# Autodesk Inventor assembly: Assembly6
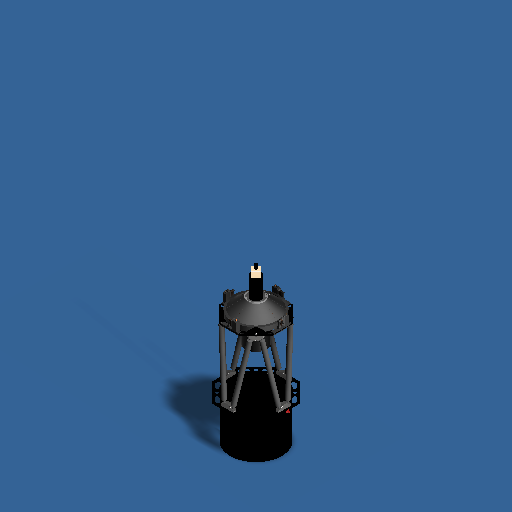
[picture p0: Inventor's stored thumbnail of the model, 512x512]
Saved by Autodesk Inventor 2026.2 (Build 302298000, 298)
## iProperties
Created: 2025-12-09
Part Number: Assembly6
Document SubType Name: Assembly
Designer: Thoma
Mass: 27295.5 g
Surface Area: 25498 cm^2
Volume: 10830.6 cm^3
Density: 2.52023 g/cm^3
Author: Thoma
## Documents named in this file (26)
- C:\Users\Thoma\OneDrive\Desktop\dir\telescope_cover\main\version_2\Main_v4.iam
- C:\Users\Thoma\OneDrive\Desktop\dir\telescope_cover\telescope\version_3\Telescope_End.ipt
- C:\Users\Thoma\OneDrive\Desktop\dir\telescope_cover\telescope\version_3\Triangle.ipt
- C:\Users\Thoma\OneDrive\Desktop\dir\telescope_cover\telescope\version_3\Triangle_Bracket_Top.ipt
- C:\Users\Thoma\OneDrive\Desktop\dir\telescope_cover\telescope\version_3\Carbon_Fibre.ipt
- C:\Users\Thoma\OneDrive\Desktop\dir\telescope_cover\telescope\version_3\5mm Screw.ipt
- C:\Users\Thoma\OneDrive\Desktop\dir\telescope_cover\telescope\version_3\35mm_bolt.ipt
- C:\Users\Thoma\OneDrive\Desktop\dir\telescope_cover\telescope\version_3\Triangle_Bracket_Bottom_MIR.ipt
- C:\Users\Thoma\OneDrive\Desktop\dir\telescope_cover\telescope\version_3\Telescope_Base.ipt
- C:\Users\Thoma\OneDrive\Desktop\dir\telescope_cover\telescope\version_3\Full_shaft_Simplify_3.ipt
- C:\Users\Thoma\OneDrive\Desktop\dir\telescope_cover\cover\Conic_Cover_Simplify_1.ipt
- C:\Users\Thoma\OneDrive\Desktop\dir\telescope_cover\telescope\version_3\30mm_bolt.ipt
- C:\Users\Thoma\OneDrive\Desktop\dir\telescope_cover\telescope\version_3\Baffle.ipt
- C:\Users\Thoma\OneDrive\Desktop\dir\telescope_cover\telescope\version_3\Bottom_End_Top.ipt
- C:\Users\Thoma\OneDrive\Desktop\dir\telescope_cover\cover\Cover_Lower_v3.ipt
- C:\Users\Thoma\OneDrive\Desktop\dir\telescope_cover\cover\Cover_Upper_v3.ipt
- C:\Users\Thoma\OneDrive\Desktop\dir\telescope_cover\telescope\version_3\Laser.ipt
- C:\Users\Thoma\OneDrive\Desktop\dir\telescope_cover\cover\rod_v10.ipt
- C:\Users\Thoma\OneDrive\Desktop\dir\telescope_cover\cover\4mm_washer_1mm.ipt
- C:\Users\Thoma\OneDrive\Desktop\dir\telescope_cover\servo\DSS-M15S Servo.ipt
- C:\Users\Thoma\OneDrive\Desktop\dir\telescope_cover\cover\Base_Plate_bottom.ipt
- C:\Users\Thoma\OneDrive\Desktop\dir\telescope_cover\cover\pawn.ipt
- C:\Users\Thoma\OneDrive\Desktop\dir\telescope_cover\cover\4mm_screw.ipt
- C:\Users\Thoma\OneDrive\Desktop\dir\telescope_cover\cover\6mm_washer_1mm.ipt
- C:\Users\Thoma\OneDrive\Desktop\dir\telescope_cover\cover\base_plate_v8.ipt
- C:\Users\Thoma\OneDrive\Desktop\dir\telescope_cover\cover\4mm_0.5_Screw.ipt
## Components (150 placed, 25 different names)
1. 30mm_bolt:9 — Mate:217, Mate:218, Angle:83
2. 30mm_bolt:10 — Mate:216, Mate:219, Angle:82
3. base_plate_v8:1 — Mate:223, Mate:227, Mate:235, Mate:238, Angle:86, Mate:244, Mate:245, Angle:91, Mate:246, Mate:249, Mate:250, Mate:293, Mate:294, Mate:295, Mate:296, Mate:297, Mate:298, Mate:299, Mate:300, Mate:301, Mate:302, Mate:303, Mate:304, Angle:104, Angle:105, Mate:308, Angle:106, Mate:310, Angle:107, Angle:127
4. base_plate_v8:2 — Mate:220, Mate:225, Mate:233, Mate:236, Angle:87, Mate:239, Mate:240, Angle:89, Mate:241, Mate:255, Mate:256, Mate:287, Mate:288, Mate:289, Mate:338, Mate:339, Mate:340, Mate:341, Mate:342, Mate:343, Mate:344, Mate:345, Mate:346, Angle:112, Mate:348, Angle:113, Mate:350, Angle:114, Mate:352, Angle:115, Angle:135
5. base_plate_v8:3 — Mate:221, Mate:226, Mate:237, Angle:88, Mate:242, Mate:243, Angle:90, Mate:247, Mate:252, Mate:253, Mate:290, Mate:291, Mate:292, Mate:354, Mate:355, Mate:356, Mate:357, Mate:358, Mate:359, Mate:360, Mate:361, Angle:116, Angle:117, Angle:118, Angle:119, Mate:385, Angle:136
6. base_plate_v8:4 — Mate:222, Mate:224, Mate:228, Mate:229, Angle:84, Mate:230, Mate:231, Angle:85, Mate:232, Mate:258, Mate:259, Mate:284, Mate:285, Mate:286, Mate:312, Mate:313, Mate:314, Mate:315, Mate:316, Mate:317, Mate:318, Mate:319, Angle:108, Angle:109, Angle:110, Angle:111, Angle:131
7. pawn:1 — Mate:228, Mate:229, Angle:84, Mate:419
8. pawn:2 — Mate:235, Mate:238, Angle:86, Mate:403
9. pawn:3 — Mate:237, Angle:88, Mate:384, Mate:386
10. pawn:4 — Mate:233, Mate:236, Angle:87, Mate:435
11. 4mm_screw:1 — Mate:230, Mate:231, Angle:85
12. 4mm_screw:2 — Mate:244, Mate:245, Angle:91
13. 4mm_screw:3 — Mate:242, Mate:243, Angle:90, Mate:385
14. 4mm_screw:4 — Mate:239, Mate:240, Angle:89
15. Base_Plate_bottom:1 — Mate:248, Mate:249, Mate:250, Mate:278, Mate:279, Angle:101, Mate:280, Mate:281, Angle:102, Mate:282, Mate:283, Angle:103
16. Base_Plate_bottom:2 — Mate:257, Mate:258, Mate:259, Mate:260, Mate:261, Mate:262, Mate:263, Angle:92, Mate:264, Angle:93, Mate:265, Angle:94
17. Base_Plate_bottom:3 — Mate:254, Mate:255, Mate:256, Mate:266, Mate:267, Angle:95, Mate:268, Mate:269, Angle:96, Mate:270, Mate:271, Angle:97
18. Base_Plate_bottom:4 — Mate:251, Mate:252, Mate:253, Mate:272, Mate:273, Angle:98, Mate:274, Mate:275, Angle:99, Mate:276, Mate:277, Angle:100
19. 4mm_screw:5 — Mate:262, Mate:263, Angle:92
20. 4mm_screw:6 — Mate:261, Mate:264, Angle:93
21. 4mm_screw:7 — Mate:260, Mate:265, Angle:94
22. 4mm_screw:8 — Mate:270, Mate:271, Angle:97
23. 4mm_screw:9 — Mate:268, Mate:269, Angle:96
24. 4mm_screw:10 — Mate:266, Mate:267, Angle:95
25. 4mm_screw:11 — Mate:276, Mate:277, Angle:100
26. 4mm_screw:12 — Mate:274, Mate:275, Angle:99
27. 4mm_screw:13 — Mate:272, Mate:273, Angle:98
28. 4mm_screw:14 — Mate:282, Mate:283, Angle:103
29. 4mm_screw:15 — Mate:280, Mate:281, Angle:102
30. 4mm_screw:16 — Mate:278, Mate:279, Angle:101
31. DSS-M15S Servo:1 — Mate:284, Mate:285, Mate:286, Mate:420
32. DSS-M15S Servo:2 — Mate:287, Mate:288, Mate:289, Mate:436
33. DSS-M15S Servo:3 — Mate:290, Mate:291, Mate:292, Mate:387, Mate:388
34. DSS-M15S Servo:4 — Mate:293, Mate:294, Mate:295, Mate:404
35. 6mm_washer_1mm:1 — Mate:299, Mate:301, Mate:306, Mate:307
36. 6mm_washer_1mm:2 — Mate:297, Mate:303, Mate:311
37. 6mm_washer_1mm:3 — Mate:296, Mate:302, Mate:309
38. 6mm_washer_1mm:4 — Mate:298, Mate:300, Mate:305
39. 4mm_screw:17 — Mate:310, Mate:311, Angle:107
40. 4mm_screw:18 — Mate:308, Mate:309, Angle:106
41. 4mm_screw:19 — Mate:306, Mate:307, Angle:105
42. 4mm_screw:20 — Mate:304, Mate:305, Angle:104
43. 6mm_washer_1mm:5 — Mate:315, Mate:317, Mate:324, Mate:325
44. 6mm_washer_1mm:6 — Mate:314, Mate:316, Mate:322, Mate:323
45. 6mm_washer_1mm:7 — Mate:313, Mate:319, Mate:326, Mate:327
46. 6mm_washer_1mm:8 — Mate:312, Mate:318, Mate:320, Mate:321
47. 4mm_screw:21 — Mate:326, Mate:327, Angle:111
48. 4mm_screw:22 — Mate:324, Mate:325, Angle:110
49. 4mm_screw:23 — Mate:322, Mate:323, Angle:109
50. 4mm_screw:24 — Mate:320, Mate:321, Angle:108
51. Cover_Lower_v3:1 — Mate:421, Mate:422, Tangent:37, Mate:429, Mate:430, Mate:431, Mate:432, Mate:433, Mate:434
52. Cover_Lower_v3:2 — Mate:389, Mate:390, Tangent:35, Mate:400, Mate:401, Mate:402
53. Cover_Upper_v3:1 — Mate:405, Mate:406, Tangent:36, Mate:413, Mate:414, Mate:415, Mate:416, Mate:417, Mate:418
54. Cover_Upper_v3:2 — Mate:370, Mate:371, Tangent:34, Mate:378, Mate:379, Mate:380, Mate:381, Mate:382, Mate:383
55. 6mm_washer_1mm:9 — Mate:341, Mate:343, Mate:349
56. 6mm_washer_1mm:10 — Mate:340, Mate:342, Mate:347
57. 6mm_washer_1mm:11 — Mate:339, Mate:345, Mate:353
58. 6mm_washer_1mm:12 — Mate:338, Mate:344, Mate:351
59. 4mm_screw:25 — Mate:350, Mate:351, Angle:114
60. 4mm_screw:26 — Mate:352, Mate:353, Angle:115
61. 4mm_screw:27 — Mate:348, Angle:113, Mate:349
62. 4mm_screw:28 — Mate:346, Mate:347, Angle:112
63. 6mm_washer_1mm:13 — Mate:360, Mate:361, Mate:364, Mate:365
64. 6mm_washer_1mm:14 — Mate:358, Mate:359, Mate:362, Mate:363
65. 6mm_washer_1mm:15 — Mate:356, Mate:357, Mate:368, Mate:369
66. 6mm_washer_1mm:16 — Mate:354, Mate:355, Mate:366, Mate:367
67. 4mm_screw:29 — Mate:368, Mate:369, Angle:119
68. 4mm_screw:30 — Mate:366, Mate:367, Angle:118
69. 4mm_screw:31 — Mate:364, Mate:365, Angle:117
70. 4mm_screw:32 — Mate:362, Mate:363, Angle:116
71. 4mm_washer_1mm:1 — Mate:376, Mate:377
72. 4mm_washer_1mm:2 — Mate:374, Mate:375
73. 4mm_washer_1mm:3 — Mate:372, Mate:373
74. 4mm_0.5_Screw:1 — Mate:378, Mate:379, Angle:121
75. 4mm_0.5_Screw:2 — Mate:382, Mate:383, Angle:122
76. 4mm_0.5_Screw:3 — Mate:380, Mate:381, Angle:120
77. 4mm_washer_1mm:4 — Mate:393, Mate:394
78. 4mm_washer_1mm:5 — Mate:392, Mate:395
79. 4mm_washer_1mm:6 — Mate:391, Mate:396
80. 4mm_0.5_Screw:4 — Mate:399, Mate:400, Angle:126
81. 4mm_0.5_Screw:5 — Mate:398, Mate:401, Angle:125
82. 4mm_0.5_Screw:6 — Mate:397, Mate:402, Angle:124
83. 4mm_washer_1mm:7 — Mate:411, Mate:412
84. 4mm_washer_1mm:8 — Mate:409, Mate:410
85. 4mm_washer_1mm:9 — Mate:407, Mate:408
86. 4mm_0.5_Screw:7 — Mate:416, Mate:417, Angle:130
87. 4mm_0.5_Screw:8 — Mate:415, Mate:418, Angle:128
88. 4mm_0.5_Screw:9 — Mate:413, Mate:414, Angle:129
89. 4mm_washer_1mm:10 — Mate:425, Mate:426
90. 4mm_washer_1mm:11 — Mate:424, Mate:427
91. 4mm_washer_1mm:12 — Mate:423, Mate:428
92. 4mm_0.5_Screw:10 — Mate:431, Mate:434, Angle:132
93. 4mm_0.5_Screw:11 — Mate:430, Mate:433, Angle:133
94. 4mm_0.5_Screw:12 — Mate:429, Mate:432, Angle:134
95. rod_v10:3 — Mate:370, Mate:371, Tangent:34, Mate:372, Mate:373, Mate:374, Mate:375, Mate:376, Mate:377, Angle:120, Angle:121, Angle:122, Mate:384, Mate:386, Mate:387, Mate:388, Angle:136
96. rod_v10:2 — Mate:405, Mate:406, Tangent:36, Mate:407, Mate:408, Mate:409, Mate:410, Mate:411, Mate:412, Angle:128, Angle:129, Angle:130, Mate:419, Mate:420, Angle:131
97. rod_v10:1 — Mate:389, Mate:390, Tangent:35, Mate:391, Mate:392, Mate:393, Mate:394, Mate:395, Mate:396, Mate:397, Mate:398, Mate:399, Angle:124, Angle:125, Angle:126, Mate:403, Mate:404, Angle:127
98. rod_v10:4 — Mate:421, Mate:422, Tangent:37, Mate:423, Mate:424, Mate:425, Mate:426, Mate:427, Mate:428, Angle:132, Angle:133, Angle:134, Mate:435, Angle:135, Mate:436
99. Laser:2 — Mate:214, Flush:220, Flush:221
100. Laser:1 — Mate:215, Flush:218, Flush:219
101. Baffle:1 — Mate:83
102. Carbon_Fibre:1 — Mate:7, Mate:11, Flush:1, Mate:12, Mate:13, Mate:14, Mate:15, Mate:62, Flush:2, Flush:3, Flush:4, Flush:5, Mate:83, Mate:92, Mate:93, Mate:96, Mate:97, Mate:98, Mate:99, Mate:100, Mate:123, Mate:124, Mate:125, Mate:213
103. Telescope_Base:1 — Mate:62, Angle:31, Mate:89, Mate:90, Angle:40, Mate:108, Mate:109, Angle:48, Mate:110, Mate:111, Angle:49, Mate:112, Mate:113, Angle:50, Mate:214, Mate:215, Flush:218, Flush:221
104. Telescope_End:1 — Mate:1, Mate:2, Angle:2, Mate:7, Mate:54, Mate:55, Angle:26, Angle:31, Mate:86, Mate:88, Mate:91, Angle:41, Mate:101, Angle:45, Angle:46, Mate:114, Mate:115, Angle:51, Mate:116, Mate:117, Angle:52, Mate:118, Mate:119, Angle:53, Mate:220, Mate:221, Mate:222, Mate:223, Mate:224, Mate:225, Mate:226, Mate:227, Mate:232, Mate:241, Mate:246, Mate:247, Mate:248, Mate:251, Mate:254, Mate:257
105. Triangle_Bracket_Top:5 — Mate:116, Mate:117, Angle:52, Mate:129, Flush:110, Angle:60
106. Triangle_Bracket_Top:4 — Mate:101, Angle:45, Angle:46, Mate:104, Mate:105, Mate:106, Flush:103, Angle:47
107. Triangle_Bracket_Top:3 — Mate:86, Mate:88, Mate:94, Angle:54, Angle:55, Mate:122, Flush:106, Angle:56
108. Triangle_Bracket_Top:1 — Mate:1, Mate:2, Angle:2, Mate:8, Mate:9, Angle:4, Mate:47, Angle:22, Mate:58
109. Triangle:1 — Mate:8, Mate:9, Angle:4, Mate:11, Flush:1, Angle:5, Angle:6, Mate:46, Mate:70, Mate:71
110. Triangle:5 — Mate:92, Mate:93, Mate:94, Mate:102, Mate:128, Flush:109, Angle:59, Mate:132, Flush:181, Angle:81
111. Triangle:6 — Mate:96, Mate:97, Mate:98, Flush:101, Angle:43, Flush:102, Angle:44, Mate:103, Mate:104, Mate:105, Mate:107
112. Triangle:7 — Mate:123, Mate:124, Mate:125, Mate:126, Flush:107, Angle:57, Mate:127, Flush:108, Angle:58, Mate:130, Mate:131
113. 35mm_bolt:6 — Mate:122, Flush:106, Angle:56
114. 35mm_bolt:7 — Mate:129, Flush:110, Angle:60
115. 35mm_bolt:4 — Mate:46, Mate:47, Angle:22
116. 35mm_bolt:5 — Mate:106, Flush:103, Angle:47
117. 5mm Screw:9 — Mate:100, Flush:102, Angle:44
118. 5mm Screw:13 — Mate:213, Flush:181, Angle:81
119. 5mm Screw:8 — Mate:99, Flush:101, Angle:43
120. 5mm Screw:10 — Mate:126, Flush:107, Angle:57
121. 5mm Screw:2 — Mate:14, Mate:15, Angle:6
122. 5mm Screw:1 — Mate:12, Mate:13, Angle:5
123. 5mm Screw:11 — Mate:127, Flush:108, Angle:58
124. 5mm Screw:12 — Mate:128, Flush:109, Angle:59
125. Full_shaft_Simplify_3:1
126. Full_shaft_Simplify_3:2 — Tangent:26
127. Full_shaft_Simplify_3:3
128. Full_shaft_Simplify_3:4
129. Full_shaft_Simplify_3:5
130. Full_shaft_Simplify_3:6
131. Full_shaft_Simplify_3:7
132. Full_shaft_Simplify_3:8 — Tangent:31, Tangent:33
133. 30mm_bolt:7 — Mate:120, Flush:104, Angle:54
134. 30mm_bolt:1 — Mate:121, Flush:105, Angle:55
135. 30mm_bolt:8 — Mate:80, Flush:13, Angle:39
136. 30mm_bolt:6 — Mate:78, Flush:11, Angle:37
137. 30mm_bolt:3 — Mate:79, Flush:12, Angle:38
138. 30mm_bolt:2 — Mate:77, Flush:10, Angle:36
139. Triangle_Bracket_Bottom_MIR:4 — Mate:118, Mate:119, Angle:53, Mate:216, Mate:217, Mate:218, Mate:219, Angle:82, Angle:83
140. Triangle_Bracket_Bottom_MIR:3 — Mate:114, Mate:115, Angle:51, Mate:120, Flush:104, Mate:121, Flush:105
141. Triangle_Bracket_Bottom_MIR:2 — Mate:55, Mate:58, Angle:26, Mate:77, Flush:10, Angle:36, Mate:78, Flush:11, Angle:37, Tangent:31
142. Triangle_Bracket_Bottom_MIR:1 — Mate:54, Mate:79, Flush:12, Angle:38, Mate:80, Flush:13, Angle:39, Mate:91, Angle:41
143. Bottom_End_Top:4 — Mate:112, Mate:113, Angle:50, Tangent:26, Tangent:33
144. Bottom_End_Top:3 — Mate:110, Mate:111, Angle:49, Flush:219
145. Bottom_End_Top:2 — Mate:108, Mate:109, Angle:48
146. Bottom_End_Top:1 — Mate:89, Mate:90, Angle:40, Flush:220
147. Conic_Cover_Simplify_1:1 — Flush:2, Mate:131, Mate:132
148. Conic_Cover_Simplify_1:2 — Flush:3, Mate:102, Mate:103
149. Conic_Cover_Simplify_1:3 — Flush:4, Mate:70, Mate:107
150. Conic_Cover_Simplify_1:4 — Mate:71, Flush:5, Mate:130
## Relationships (398: Mate 281, Angle 86, Flush 24, Tangent 7)
- Mate:1: Telescope_End:1 ↔ Triangle_Bracket_Top:1
- Mate:2: Telescope_End:1 ↔ Triangle_Bracket_Top:1
- Angle:2 (0 deg): Telescope_End:1 ↔ Triangle_Bracket_Top:1
- Mate:7: Carbon_Fibre:1 ↔ Telescope_End:1
- Mate:8: Triangle_Bracket_Top:1 ↔ Triangle:1
- Mate:9: Triangle_Bracket_Top:1 ↔ Triangle:1
- Angle:4 (0 deg): Triangle_Bracket_Top:1 ↔ Triangle:1
- Mate:11: Carbon_Fibre:1 ↔ Triangle:1
- Flush:1: Carbon_Fibre:1 ↔ Triangle:1
- Mate:12: Carbon_Fibre:1 ↔ 5mm Screw:1
- Mate:13: Carbon_Fibre:1 ↔ 5mm Screw:1
- Angle:5 (0 deg): Triangle:1 ↔ 5mm Screw:1
- Mate:14: Carbon_Fibre:1 ↔ 5mm Screw:2
- Mate:15: Carbon_Fibre:1 ↔ 5mm Screw:2
- Angle:6 (0 deg): Triangle:1 ↔ 5mm Screw:2
- Mate:46: Triangle:1 ↔ 35mm_bolt:4
- Mate:47: Triangle_Bracket_Top:1 ↔ 35mm_bolt:4
- Angle:22 (0 deg): Triangle_Bracket_Top:1 ↔ 35mm_bolt:4
- Mate:54: Telescope_End:1 ↔ Triangle_Bracket_Bottom_MIR:1
- Mate:55: Telescope_End:1 ↔ Triangle_Bracket_Bottom_MIR:2
- Mate:58: Triangle_Bracket_Top:1 ↔ Triangle_Bracket_Bottom_MIR:2
- Angle:26 (0 deg): Telescope_End:1 ↔ Triangle_Bracket_Bottom_MIR:2
- Mate:62: Carbon_Fibre:1 ↔ Telescope_Base:1
- Angle:31 (0 deg): Telescope_Base:1 ↔ Telescope_End:1
- Flush:2: Carbon_Fibre:1 ↔ Conic_Cover_Simplify_1:1
- Flush:3: Carbon_Fibre:1 ↔ Conic_Cover_Simplify_1:2
- Flush:4: Carbon_Fibre:1 ↔ Conic_Cover_Simplify_1:3
- Mate:70: Triangle:1 ↔ Conic_Cover_Simplify_1:3
- Mate:71: Triangle:1 ↔ Conic_Cover_Simplify_1:4
- Flush:5: Carbon_Fibre:1 ↔ Conic_Cover_Simplify_1:4
- Mate:77: 30mm_bolt:2 ↔ Triangle_Bracket_Bottom_MIR:2
- Flush:10: 30mm_bolt:2 ↔ Triangle_Bracket_Bottom_MIR:2
- Angle:36 (0 deg): 30mm_bolt:2 ↔ Triangle_Bracket_Bottom_MIR:2
- Mate:78: 30mm_bolt:6 ↔ Triangle_Bracket_Bottom_MIR:2
- Flush:11: 30mm_bolt:6 ↔ Triangle_Bracket_Bottom_MIR:2
- Angle:37 (0 deg): 30mm_bolt:6 ↔ Triangle_Bracket_Bottom_MIR:2
- Mate:79: 30mm_bolt:3 ↔ Triangle_Bracket_Bottom_MIR:1
- Flush:12: 30mm_bolt:3 ↔ Triangle_Bracket_Bottom_MIR:1
- Angle:38 (0 deg): 30mm_bolt:3 ↔ Triangle_Bracket_Bottom_MIR:1
- Mate:80: 30mm_bolt:8 ↔ Triangle_Bracket_Bottom_MIR:1
- Flush:13: 30mm_bolt:8 ↔ Triangle_Bracket_Bottom_MIR:1
- Angle:39 (0 deg): 30mm_bolt:8 ↔ Triangle_Bracket_Bottom_MIR:1
- Mate:83: Baffle:1 ↔ Carbon_Fibre:1
- Mate:86: Telescope_End:1 ↔ Triangle_Bracket_Top:3
- Mate:88: Telescope_End:1 ↔ Triangle_Bracket_Top:3
- Mate:89: Telescope_Base:1 ↔ Bottom_End_Top:1
- Mate:90: Telescope_Base:1 ↔ Bottom_End_Top:1
- Angle:40 (0 deg): Telescope_Base:1 ↔ Bottom_End_Top:1
- Mate:91: Telescope_End:1 ↔ Triangle_Bracket_Bottom_MIR:1
- Angle:41 (0 deg): Telescope_End:1 ↔ Triangle_Bracket_Bottom_MIR:1
- Mate:92: Carbon_Fibre:1 ↔ Triangle:5
- Mate:93: Carbon_Fibre:1 ↔ Triangle:5
- Mate:94: Triangle_Bracket_Top:3 ↔ Triangle:5
- Mate:96: Carbon_Fibre:1 ↔ Triangle:6
- Mate:97: Carbon_Fibre:1 ↔ Triangle:6
- Mate:98: Carbon_Fibre:1 ↔ Triangle:6
- Mate:99: Carbon_Fibre:1 ↔ 5mm Screw:8
- Flush:101: Triangle:6 ↔ 5mm Screw:8
- Angle:43 (0 deg): Triangle:6 ↔ 5mm Screw:8
- Mate:100: Carbon_Fibre:1 ↔ 5mm Screw:9
- Flush:102: Triangle:6 ↔ 5mm Screw:9
- Angle:44 (0 deg): Triangle:6 ↔ 5mm Screw:9
- Mate:101: Telescope_End:1 ↔ Triangle_Bracket_Top:4
- Angle:45 (0 deg): Telescope_End:1 ↔ Triangle_Bracket_Top:4
- Mate:102: Triangle:5 ↔ Conic_Cover_Simplify_1:2
- Mate:103: Triangle:6 ↔ Conic_Cover_Simplify_1:2
- Angle:46 (0 deg): Telescope_End:1 ↔ Triangle_Bracket_Top:4
- Mate:104: Triangle_Bracket_Top:4 ↔ Triangle:6
- Mate:105: Triangle_Bracket_Top:4 ↔ Triangle:6
- Mate:106: Triangle_Bracket_Top:4 ↔ 35mm_bolt:5
- Flush:103: Triangle_Bracket_Top:4 ↔ 35mm_bolt:5
- Angle:47 (0 deg): Triangle_Bracket_Top:4 ↔ 35mm_bolt:5
- Mate:107: Triangle:6 ↔ Conic_Cover_Simplify_1:3
- Mate:108: Telescope_Base:1 ↔ Bottom_End_Top:2
- Mate:109: Telescope_Base:1 ↔ Bottom_End_Top:2
- Angle:48 (0 deg): Telescope_Base:1 ↔ Bottom_End_Top:2
- Mate:110: Telescope_Base:1 ↔ Bottom_End_Top:3
- Mate:111: Telescope_Base:1 ↔ Bottom_End_Top:3
- Angle:49 (0 deg): Telescope_Base:1 ↔ Bottom_End_Top:3
- Mate:112: Telescope_Base:1 ↔ Bottom_End_Top:4
- Mate:113: Telescope_Base:1 ↔ Bottom_End_Top:4
- Angle:50 (0 deg): Telescope_Base:1 ↔ Bottom_End_Top:4
- Mate:114: Telescope_End:1 ↔ Triangle_Bracket_Bottom_MIR:3
- Mate:115: Telescope_End:1 ↔ Triangle_Bracket_Bottom_MIR:3
- Angle:51 (0 deg): Telescope_End:1 ↔ Triangle_Bracket_Bottom_MIR:3
- Mate:116: Telescope_End:1 ↔ Triangle_Bracket_Top:5
- Mate:117: Telescope_End:1 ↔ Triangle_Bracket_Top:5
- Angle:52 (0 deg): Telescope_End:1 ↔ Triangle_Bracket_Top:5
- Mate:118: Telescope_End:1 ↔ Triangle_Bracket_Bottom_MIR:4
- Mate:119: Telescope_End:1 ↔ Triangle_Bracket_Bottom_MIR:4
- Angle:53 (0 deg): Telescope_End:1 ↔ Triangle_Bracket_Bottom_MIR:4
- Mate:120: 30mm_bolt:7 ↔ Triangle_Bracket_Bottom_MIR:3
- Flush:104: 30mm_bolt:7 ↔ Triangle_Bracket_Bottom_MIR:3
- Angle:54 (0 deg): Triangle_Bracket_Top:3 ↔ 30mm_bolt:7
- Mate:121: 30mm_bolt:1 ↔ Triangle_Bracket_Bottom_MIR:3
- Flush:105: 30mm_bolt:1 ↔ Triangle_Bracket_Bottom_MIR:3
- Angle:55 (0 deg): Triangle_Bracket_Top:3 ↔ 30mm_bolt:1
- Mate:122: Triangle_Bracket_Top:3 ↔ 35mm_bolt:6
- Flush:106: Triangle_Bracket_Top:3 ↔ 35mm_bolt:6
- Angle:56 (0 deg): Triangle_Bracket_Top:3 ↔ 35mm_bolt:6
- Mate:123: Carbon_Fibre:1 ↔ Triangle:7
- Mate:124: Carbon_Fibre:1 ↔ Triangle:7
- Mate:125: Carbon_Fibre:1 ↔ Triangle:7
- Mate:126: Triangle:7 ↔ 5mm Screw:10
- Flush:107: Triangle:7 ↔ 5mm Screw:10
- Angle:57 (0 deg): Triangle:7 ↔ 5mm Screw:10
- Mate:127: Triangle:7 ↔ 5mm Screw:11
- Flush:108: Triangle:7 ↔ 5mm Screw:11
- Angle:58 (0 deg): Triangle:7 ↔ 5mm Screw:11
- Mate:128: Triangle:5 ↔ 5mm Screw:12
- Flush:109: Triangle:5 ↔ 5mm Screw:12
- Angle:59 (0 deg): Triangle:5 ↔ 5mm Screw:12
- Mate:129: Triangle_Bracket_Top:5 ↔ 35mm_bolt:7
- Flush:110: Triangle_Bracket_Top:5 ↔ 35mm_bolt:7
- Angle:60 (0 deg): Triangle_Bracket_Top:5 ↔ 35mm_bolt:7
- Mate:130: Triangle:7 ↔ Conic_Cover_Simplify_1:4
- Mate:131: Triangle:7 ↔ Conic_Cover_Simplify_1:1
- Mate:132: Triangle:5 ↔ Conic_Cover_Simplify_1:1
- Mate:213: Carbon_Fibre:1 ↔ 5mm Screw:13
- Flush:181: Triangle:5 ↔ 5mm Screw:13
- Angle:81 (0 deg): Triangle:5 ↔ 5mm Screw:13
- Mate:214: Laser:2 ↔ Telescope_Base:1
- Mate:215: Laser:1 ↔ Telescope_Base:1
- Flush:218: Laser:1 ↔ Telescope_Base:1
- Flush:219 (39.316 mm): Laser:1 ↔ Bottom_End_Top:3
- Flush:220 (39.316 mm): Laser:2 ↔ Bottom_End_Top:1
- Flush:221: Laser:2 ↔ Telescope_Base:1
- Tangent:26: Full_shaft_Simplify_3:2 ↔ Bottom_End_Top:4
- Tangent:31: Full_shaft_Simplify_3:8 ↔ Triangle_Bracket_Bottom_MIR:2
- Tangent:33: Full_shaft_Simplify_3:8 ↔ Bottom_End_Top:4
- Mate:216: 30mm_bolt:10 ↔ Triangle_Bracket_Bottom_MIR:4
- Mate:217: 30mm_bolt:9 ↔ Triangle_Bracket_Bottom_MIR:4
- Mate:218: 30mm_bolt:9 ↔ Triangle_Bracket_Bottom_MIR:4
- Mate:219: 30mm_bolt:10 ↔ Triangle_Bracket_Bottom_MIR:4
- Angle:82 (0 deg): 30mm_bolt:10 ↔ Triangle_Bracket_Bottom_MIR:4
- Angle:83 (0 deg): 30mm_bolt:9 ↔ Triangle_Bracket_Bottom_MIR:4
- Mate:220: base_plate_v8:2 ↔ Telescope_End:1
- Mate:221: base_plate_v8:3 ↔ Telescope_End:1
- Mate:222: base_plate_v8:4 ↔ Telescope_End:1
- Mate:223: base_plate_v8:1 ↔ Telescope_End:1
- Mate:224: base_plate_v8:4 ↔ Telescope_End:1
- Mate:225: base_plate_v8:2 ↔ Telescope_End:1
- Mate:226: base_plate_v8:3 ↔ Telescope_End:1
- Mate:227: base_plate_v8:1 ↔ Telescope_End:1
- Mate:228: base_plate_v8:4 ↔ pawn:1
- Mate:229: base_plate_v8:4 ↔ pawn:1
- Angle:84 (180 deg): base_plate_v8:4 ↔ pawn:1
- Mate:230: base_plate_v8:4 ↔ 4mm_screw:1
- Mate:231: base_plate_v8:4 ↔ 4mm_screw:1
- Angle:85 (0 deg): base_plate_v8:4 ↔ 4mm_screw:1
- Mate:232: base_plate_v8:4 ↔ Telescope_End:1
- Mate:233: base_plate_v8:2 ↔ pawn:4
- Mate:235: base_plate_v8:1 ↔ pawn:2
- Mate:236: base_plate_v8:2 ↔ pawn:4
- Mate:237: base_plate_v8:3 ↔ pawn:3
- Mate:238: base_plate_v8:1 ↔ pawn:2
- Angle:86 (0 deg): base_plate_v8:1 ↔ pawn:2
- Angle:87 (0 deg): base_plate_v8:2 ↔ pawn:4
- Angle:88 (0 deg): base_plate_v8:3 ↔ pawn:3
- Mate:239: base_plate_v8:2 ↔ 4mm_screw:4
- Mate:240: base_plate_v8:2 ↔ 4mm_screw:4
- Angle:89 (0 deg): base_plate_v8:2 ↔ 4mm_screw:4
- Mate:241: base_plate_v8:2 ↔ Telescope_End:1
- Mate:242: base_plate_v8:3 ↔ 4mm_screw:3
- Mate:243: base_plate_v8:3 ↔ 4mm_screw:3
- Angle:90 (0 deg): base_plate_v8:3 ↔ 4mm_screw:3
- Mate:244: base_plate_v8:1 ↔ 4mm_screw:2
- Mate:245: base_plate_v8:1 ↔ 4mm_screw:2
- Angle:91 (0 deg): base_plate_v8:1 ↔ 4mm_screw:2
- Mate:246: base_plate_v8:1 ↔ Telescope_End:1
- Mate:247: base_plate_v8:3 ↔ Telescope_End:1
- Mate:248: Base_Plate_bottom:1 ↔ Telescope_End:1
- Mate:249: base_plate_v8:1 ↔ Base_Plate_bottom:1
- Mate:250: base_plate_v8:1 ↔ Base_Plate_bottom:1
- Mate:251: Base_Plate_bottom:4 ↔ Telescope_End:1
- Mate:252: base_plate_v8:3 ↔ Base_Plate_bottom:4
- Mate:253: base_plate_v8:3 ↔ Base_Plate_bottom:4
- Mate:254: Base_Plate_bottom:3 ↔ Telescope_End:1
- Mate:255: base_plate_v8:2 ↔ Base_Plate_bottom:3
- Mate:256: base_plate_v8:2 ↔ Base_Plate_bottom:3
- Mate:257: Base_Plate_bottom:2 ↔ Telescope_End:1
- Mate:258: base_plate_v8:4 ↔ Base_Plate_bottom:2
- Mate:259: base_plate_v8:4 ↔ Base_Plate_bottom:2
- Mate:260: Base_Plate_bottom:2 ↔ 4mm_screw:7
- Mate:261: Base_Plate_bottom:2 ↔ 4mm_screw:6
- Mate:262: Base_Plate_bottom:2 ↔ 4mm_screw:5
- Mate:263: Base_Plate_bottom:2 ↔ 4mm_screw:5
- Angle:92 (0 deg): Base_Plate_bottom:2 ↔ 4mm_screw:5
- Mate:264: Base_Plate_bottom:2 ↔ 4mm_screw:6
- Angle:93 (0 deg): Base_Plate_bottom:2 ↔ 4mm_screw:6
- Mate:265: Base_Plate_bottom:2 ↔ 4mm_screw:7
- Angle:94 (0 deg): Base_Plate_bottom:2 ↔ 4mm_screw:7
- Mate:266: Base_Plate_bottom:3 ↔ 4mm_screw:10
- Mate:267: Base_Plate_bottom:3 ↔ 4mm_screw:10
- Angle:95 (0 deg): Base_Plate_bottom:3 ↔ 4mm_screw:10
- Mate:268: Base_Plate_bottom:3 ↔ 4mm_screw:9
- Mate:269: Base_Plate_bottom:3 ↔ 4mm_screw:9
- Angle:96 (0 deg): Base_Plate_bottom:3 ↔ 4mm_screw:9
- Mate:270: Base_Plate_bottom:3 ↔ 4mm_screw:8
- Mate:271: Base_Plate_bottom:3 ↔ 4mm_screw:8
- Angle:97 (0 deg): Base_Plate_bottom:3 ↔ 4mm_screw:8
- Mate:272: Base_Plate_bottom:4 ↔ 4mm_screw:13
- Mate:273: Base_Plate_bottom:4 ↔ 4mm_screw:13
- Angle:98 (0 deg): Base_Plate_bottom:4 ↔ 4mm_screw:13
- Mate:274: Base_Plate_bottom:4 ↔ 4mm_screw:12
- Mate:275: Base_Plate_bottom:4 ↔ 4mm_screw:12
- Angle:99 (0 deg): Base_Plate_bottom:4 ↔ 4mm_screw:12
- Mate:276: Base_Plate_bottom:4 ↔ 4mm_screw:11
- Mate:277: Base_Plate_bottom:4 ↔ 4mm_screw:11
- Angle:100 (0 deg): Base_Plate_bottom:4 ↔ 4mm_screw:11
- Mate:278: Base_Plate_bottom:1 ↔ 4mm_screw:16
- Mate:279: Base_Plate_bottom:1 ↔ 4mm_screw:16
- Angle:101 (0 deg): Base_Plate_bottom:1 ↔ 4mm_screw:16
- Mate:280: Base_Plate_bottom:1 ↔ 4mm_screw:15
- Mate:281: Base_Plate_bottom:1 ↔ 4mm_screw:15
- Angle:102 (0 deg): Base_Plate_bottom:1 ↔ 4mm_screw:15
- Mate:282: Base_Plate_bottom:1 ↔ 4mm_screw:14
- Mate:283: Base_Plate_bottom:1 ↔ 4mm_screw:14
- Angle:103 (0 deg): Base_Plate_bottom:1 ↔ 4mm_screw:14
- Mate:284 (1.1 mm): base_plate_v8:4 ↔ DSS-M15S Servo:1
- Mate:285: base_plate_v8:4 ↔ DSS-M15S Servo:1
- Mate:286: base_plate_v8:4 ↔ DSS-M15S Servo:1
- Mate:287 (1.1 mm): base_plate_v8:2 ↔ DSS-M15S Servo:2
- Mate:288: base_plate_v8:2 ↔ DSS-M15S Servo:2
- Mate:289: base_plate_v8:2 ↔ DSS-M15S Servo:2
- Mate:290 (1.1 mm): base_plate_v8:3 ↔ DSS-M15S Servo:3
- Mate:291: base_plate_v8:3 ↔ DSS-M15S Servo:3
- Mate:292: base_plate_v8:3 ↔ DSS-M15S Servo:3
- Mate:293 (1.1 mm): base_plate_v8:1 ↔ DSS-M15S Servo:4
- Mate:294: base_plate_v8:1 ↔ DSS-M15S Servo:4
- Mate:295: base_plate_v8:1 ↔ DSS-M15S Servo:4
- Mate:296: base_plate_v8:1 ↔ 6mm_washer_1mm:3
- Mate:297: base_plate_v8:1 ↔ 6mm_washer_1mm:2
- Mate:298: base_plate_v8:1 ↔ 6mm_washer_1mm:4
- Mate:299: base_plate_v8:1 ↔ 6mm_washer_1mm:1
- Mate:300: base_plate_v8:1 ↔ 6mm_washer_1mm:4
- Mate:301: base_plate_v8:1 ↔ 6mm_washer_1mm:1
- Mate:302: base_plate_v8:1 ↔ 6mm_washer_1mm:3
- Mate:303: base_plate_v8:1 ↔ 6mm_washer_1mm:2
- Mate:304: base_plate_v8:1 ↔ 4mm_screw:20
- Mate:305: 6mm_washer_1mm:4 ↔ 4mm_screw:20
- Angle:104 (0 deg): base_plate_v8:1 ↔ 4mm_screw:20
- Mate:306: 6mm_washer_1mm:1 ↔ 4mm_screw:19
- Mate:307: 6mm_washer_1mm:1 ↔ 4mm_screw:19
- Angle:105 (0 deg): base_plate_v8:1 ↔ 4mm_screw:19
- Mate:308: base_plate_v8:1 ↔ 4mm_screw:18
- Mate:309: 6mm_washer_1mm:3 ↔ 4mm_screw:18
- Angle:106 (0 deg): base_plate_v8:1 ↔ 4mm_screw:18
- Mate:310: base_plate_v8:1 ↔ 4mm_screw:17
- Mate:311: 6mm_washer_1mm:2 ↔ 4mm_screw:17
- Angle:107 (0 deg): base_plate_v8:1 ↔ 4mm_screw:17
- Mate:312: base_plate_v8:4 ↔ 6mm_washer_1mm:8
- Mate:313: base_plate_v8:4 ↔ 6mm_washer_1mm:7
- Mate:314: base_plate_v8:4 ↔ 6mm_washer_1mm:6
- Mate:315: base_plate_v8:4 ↔ 6mm_washer_1mm:5
- Mate:316: base_plate_v8:4 ↔ 6mm_washer_1mm:6
- Mate:317: base_plate_v8:4 ↔ 6mm_washer_1mm:5
- Mate:318: base_plate_v8:4 ↔ 6mm_washer_1mm:8
- Mate:319: base_plate_v8:4 ↔ 6mm_washer_1mm:7
- Mate:320: 6mm_washer_1mm:8 ↔ 4mm_screw:24
- Mate:321: 6mm_washer_1mm:8 ↔ 4mm_screw:24
- Angle:108 (0 deg): base_plate_v8:4 ↔ 4mm_screw:24
- Mate:322: 6mm_washer_1mm:6 ↔ 4mm_screw:23
- Mate:323: 6mm_washer_1mm:6 ↔ 4mm_screw:23
- Angle:109 (0 deg): base_plate_v8:4 ↔ 4mm_screw:23
- Mate:324: 6mm_washer_1mm:5 ↔ 4mm_screw:22
- Mate:325: 6mm_washer_1mm:5 ↔ 4mm_screw:22
- Angle:110 (0 deg): base_plate_v8:4 ↔ 4mm_screw:22
- Mate:326: 6mm_washer_1mm:7 ↔ 4mm_screw:21
- Mate:327: 6mm_washer_1mm:7 ↔ 4mm_screw:21
- Angle:111 (0 deg): base_plate_v8:4 ↔ 4mm_screw:21
- Mate:338: base_plate_v8:2 ↔ 6mm_washer_1mm:12
- Mate:339: base_plate_v8:2 ↔ 6mm_washer_1mm:11
- Mate:340: base_plate_v8:2 ↔ 6mm_washer_1mm:10
- Mate:341: base_plate_v8:2 ↔ 6mm_washer_1mm:9
- Mate:342: base_plate_v8:2 ↔ 6mm_washer_1mm:10
- Mate:343: base_plate_v8:2 ↔ 6mm_washer_1mm:9
- Mate:344: base_plate_v8:2 ↔ 6mm_washer_1mm:12
- Mate:345: base_plate_v8:2 ↔ 6mm_washer_1mm:11
- Mate:346: base_plate_v8:2 ↔ 4mm_screw:28
- Mate:347: 6mm_washer_1mm:10 ↔ 4mm_screw:28
- Angle:112 (0 deg): base_plate_v8:2 ↔ 4mm_screw:28
- Mate:348: base_plate_v8:2 ↔ 4mm_screw:27
- Angle:113 (0 deg): base_plate_v8:2 ↔ 4mm_screw:27
- Mate:349: 6mm_washer_1mm:9 ↔ 4mm_screw:27
- Mate:350: base_plate_v8:2 ↔ 4mm_screw:25
- Mate:351: 6mm_washer_1mm:12 ↔ 4mm_screw:25
- Angle:114 (0 deg): base_plate_v8:2 ↔ 4mm_screw:25
- Mate:352: base_plate_v8:2 ↔ 4mm_screw:26
- Mate:353: 6mm_washer_1mm:11 ↔ 4mm_screw:26
- Angle:115 (0 deg): base_plate_v8:2 ↔ 4mm_screw:26
- Mate:354: base_plate_v8:3 ↔ 6mm_washer_1mm:16
- Mate:355: base_plate_v8:3 ↔ 6mm_washer_1mm:16
- Mate:356: base_plate_v8:3 ↔ 6mm_washer_1mm:15
- Mate:357: base_plate_v8:3 ↔ 6mm_washer_1mm:15
- Mate:358: base_plate_v8:3 ↔ 6mm_washer_1mm:14
- Mate:359: base_plate_v8:3 ↔ 6mm_washer_1mm:14
- Mate:360: base_plate_v8:3 ↔ 6mm_washer_1mm:13
- Mate:361: base_plate_v8:3 ↔ 6mm_washer_1mm:13
- Mate:362: 6mm_washer_1mm:14 ↔ 4mm_screw:32
- Mate:363: 6mm_washer_1mm:14 ↔ 4mm_screw:32
- Angle:116 (0 deg): base_plate_v8:3 ↔ 4mm_screw:32
- Mate:364: 6mm_washer_1mm:13 ↔ 4mm_screw:31
- Mate:365: 6mm_washer_1mm:13 ↔ 4mm_screw:31
- Angle:117 (0 deg): base_plate_v8:3 ↔ 4mm_screw:31
- Mate:366: 6mm_washer_1mm:16 ↔ 4mm_screw:30
- Mate:367: 6mm_washer_1mm:16 ↔ 4mm_screw:30
- Angle:118 (0 deg): base_plate_v8:3 ↔ 4mm_screw:30
- Mate:368: 6mm_washer_1mm:15 ↔ 4mm_screw:29
- Mate:369: 6mm_washer_1mm:15 ↔ 4mm_screw:29
- Angle:119 (0 deg): base_plate_v8:3 ↔ 4mm_screw:29
- Mate:370: Cover_Upper_v3:2 ↔ rod_v10:3
- Mate:371: Cover_Upper_v3:2 ↔ rod_v10:3
- Tangent:34 (-1 mm): Cover_Upper_v3:2 ↔ rod_v10:3
- Mate:372: 4mm_washer_1mm:3 ↔ rod_v10:3
- Mate:373: 4mm_washer_1mm:3 ↔ rod_v10:3
- Mate:374: 4mm_washer_1mm:2 ↔ rod_v10:3
- Mate:375: 4mm_washer_1mm:2 ↔ rod_v10:3
- Mate:376: 4mm_washer_1mm:1 ↔ rod_v10:3
- Mate:377: 4mm_washer_1mm:1 ↔ rod_v10:3
- Mate:378: Cover_Upper_v3:2 ↔ 4mm_0.5_Screw:1
- Mate:379: Cover_Upper_v3:2 ↔ 4mm_0.5_Screw:1
- Mate:380: Cover_Upper_v3:2 ↔ 4mm_0.5_Screw:3
- Mate:381: Cover_Upper_v3:2 ↔ 4mm_0.5_Screw:3
- Angle:120 (0 deg): 4mm_0.5_Screw:3 ↔ rod_v10:3
- Angle:121 (0 deg): 4mm_0.5_Screw:1 ↔ rod_v10:3
- Mate:382: Cover_Upper_v3:2 ↔ 4mm_0.5_Screw:2
- Mate:383: Cover_Upper_v3:2 ↔ 4mm_0.5_Screw:2
- Angle:122 (0 deg): 4mm_0.5_Screw:2 ↔ rod_v10:3
- Mate:384: pawn:3 ↔ rod_v10:3
- Mate:385: base_plate_v8:3 ↔ 4mm_screw:3
- Mate:386: pawn:3 ↔ rod_v10:3
- Mate:387: DSS-M15S Servo:3 ↔ rod_v10:3
- Mate:388: DSS-M15S Servo:3 ↔ rod_v10:3
- Mate:389: Cover_Lower_v3:2 ↔ rod_v10:1
- Mate:390: Cover_Lower_v3:2 ↔ rod_v10:1
- Tangent:35 (-1 mm): Cover_Lower_v3:2 ↔ rod_v10:1
- Mate:391: 4mm_washer_1mm:6 ↔ rod_v10:1
- Mate:392: 4mm_washer_1mm:5 ↔ rod_v10:1
- Mate:393: 4mm_washer_1mm:4 ↔ rod_v10:1
- Mate:394: 4mm_washer_1mm:4 ↔ rod_v10:1
- Mate:395: 4mm_washer_1mm:5 ↔ rod_v10:1
- Mate:396: 4mm_washer_1mm:6 ↔ rod_v10:1
- Mate:397: 4mm_0.5_Screw:6 ↔ rod_v10:1
- Mate:398: 4mm_0.5_Screw:5 ↔ rod_v10:1
- Mate:399: 4mm_0.5_Screw:4 ↔ rod_v10:1
- Mate:400: Cover_Lower_v3:2 ↔ 4mm_0.5_Screw:4
- Mate:401: Cover_Lower_v3:2 ↔ 4mm_0.5_Screw:5
- Mate:402: Cover_Lower_v3:2 ↔ 4mm_0.5_Screw:6
- Angle:124 (0 deg): 4mm_0.5_Screw:6 ↔ rod_v10:1
- Angle:125 (0 deg): 4mm_0.5_Screw:5 ↔ rod_v10:1
- Angle:126 (0 deg): 4mm_0.5_Screw:4 ↔ rod_v10:1
- Mate:403: pawn:2 ↔ rod_v10:1
- Mate:404: DSS-M15S Servo:4 ↔ rod_v10:1
- Angle:127 (232.647 deg): base_plate_v8:1 ↔ rod_v10:1
- Mate:405: Cover_Upper_v3:1 ↔ rod_v10:2
- Mate:406: Cover_Upper_v3:1 ↔ rod_v10:2
- Tangent:36 (-1 mm): Cover_Upper_v3:1 ↔ rod_v10:2
- Mate:407: 4mm_washer_1mm:9 ↔ rod_v10:2
- Mate:408: 4mm_washer_1mm:9 ↔ rod_v10:2
- Mate:409: 4mm_washer_1mm:8 ↔ rod_v10:2
- Mate:410: 4mm_washer_1mm:8 ↔ rod_v10:2
- Mate:411: 4mm_washer_1mm:7 ↔ rod_v10:2
- Mate:412: 4mm_washer_1mm:7 ↔ rod_v10:2
- Mate:413: Cover_Upper_v3:1 ↔ 4mm_0.5_Screw:9
- Mate:414: Cover_Upper_v3:1 ↔ 4mm_0.5_Screw:9
- Mate:415: Cover_Upper_v3:1 ↔ 4mm_0.5_Screw:8
- Mate:416: Cover_Upper_v3:1 ↔ 4mm_0.5_Screw:7
- Mate:417: Cover_Upper_v3:1 ↔ 4mm_0.5_Screw:7
- Mate:418: Cover_Upper_v3:1 ↔ 4mm_0.5_Screw:8
- Angle:128 (0 deg): 4mm_0.5_Screw:8 ↔ rod_v10:2
- Angle:129 (0 deg): 4mm_0.5_Screw:9 ↔ rod_v10:2
- Angle:130 (0 deg): 4mm_0.5_Screw:7 ↔ rod_v10:2
- Mate:419: pawn:1 ↔ rod_v10:2
- Mate:420: DSS-M15S Servo:1 ↔ rod_v10:2
- Angle:131 (127.357 deg): base_plate_v8:4 ↔ rod_v10:2
- Mate:421: Cover_Lower_v3:1 ↔ rod_v10:4
- Mate:422: Cover_Lower_v3:1 ↔ rod_v10:4
- Tangent:37 (-1 mm): Cover_Lower_v3:1 ↔ rod_v10:4
- Mate:423: 4mm_washer_1mm:12 ↔ rod_v10:4
- Mate:424: 4mm_washer_1mm:11 ↔ rod_v10:4
- Mate:425: 4mm_washer_1mm:10 ↔ rod_v10:4
- Mate:426: 4mm_washer_1mm:10 ↔ rod_v10:4
- Mate:427: 4mm_washer_1mm:11 ↔ rod_v10:4
- Mate:428: 4mm_washer_1mm:12 ↔ rod_v10:4
- Mate:429: Cover_Lower_v3:1 ↔ 4mm_0.5_Screw:12
- Mate:430: Cover_Lower_v3:1 ↔ 4mm_0.5_Screw:11
- Mate:431: Cover_Lower_v3:1 ↔ 4mm_0.5_Screw:10
- Mate:432: Cover_Lower_v3:1 ↔ 4mm_0.5_Screw:12
- Mate:433: Cover_Lower_v3:1 ↔ 4mm_0.5_Screw:11
- Mate:434: Cover_Lower_v3:1 ↔ 4mm_0.5_Screw:10
- Angle:132 (0 deg): 4mm_0.5_Screw:10 ↔ rod_v10:4
- Angle:133 (0 deg): 4mm_0.5_Screw:11 ↔ rod_v10:4
- Angle:134 (0 deg): 4mm_0.5_Screw:12 ↔ rod_v10:4
- Mate:435: pawn:4 ↔ rod_v10:4
- Angle:135 (127.357 deg): base_plate_v8:2 ↔ rod_v10:4
- Mate:436: DSS-M15S Servo:2 ↔ rod_v10:4
- Angle:136 (127.357 deg): base_plate_v8:3 ↔ rod_v10:3
